# Autodesk Inventor assembly: Assembly completo cajon gde
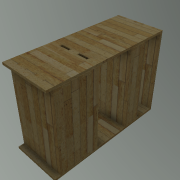
[picture p0: Inventor's stored thumbnail of the model, 180x180]
Saved by Autodesk Inventor 2015 (Build 190159000, 159)
## iProperties
Created: 2016-01-28
Part Number: Assembly completo cajon gde
Document SubType Name: Assembly
Designer: 172406
Author: 172406
## Documents named in this file (4)
- H:\3d\Assembly completo cajon gde.iam
- H:\3d\Assembly cajon grande.iam
- H:\3d\Assembly cajon.iam
- H:\3d\Assembly mueble cajon gde.iam
## Components (3 placed, 3 different names)
1. Assembly cajon grande:1 [sub-assembly] — Mate:2, Flush:1, Mate:4
2. Assembly cajon:1 [sub-assembly] — Mate:1, Flush:2, Mate:3
3. Assembly mueble cajon gde:1 [sub-assembly] — Mate:1, Mate:2, Flush:1, Flush:2, Mate:3, Mate:4
## Relationships (6: Mate 4, Flush 2)
- Mate:1: Assembly cajon:1 ↔ Assembly mueble cajon gde:1
- Mate:2: Assembly cajon grande:1 ↔ Assembly mueble cajon gde:1
- Flush:1: Assembly cajon grande:1 ↔ Assembly mueble cajon gde:1
- Flush:2: Assembly cajon:1 ↔ Assembly mueble cajon gde:1
- Mate:3 (2 mm): Assembly cajon:1 ↔ Assembly mueble cajon gde:1
- Mate:4 (2 mm): Assembly cajon grande:1 ↔ Assembly mueble cajon gde:1
